# Autodesk Inventor assembly: RR-PCSS-2021-W2M1
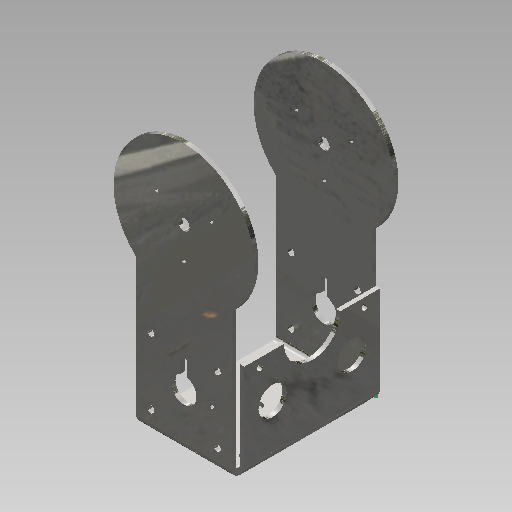
[picture p0: Inventor's stored thumbnail of the model, 512x512]
Saved by Autodesk Inventor 2021 (Build 250183000, 183)
## iProperties
Created: 2021-10-12
Part Number: RR-PCSS-2021-W2M1
Document SubType Name: Assembly
Designer: marci
Mass: 985.997 g
Surface Area: 877.416 cm^2
Volume: 123.25 cm^3
Density: 8 g/cm^3
Author: marci
## Documents named in this file (3)
- C:\Users\marci\Desktop\Projekt ramienia\2M1\RR-PCSS-2021-W2M1.iam
- C:\Users\marci\Desktop\Projekt ramienia\2M1\RR-PCSS-2021-W2M1Dn.ipt
- C:\Users\marci\Desktop\Projekt ramienia\2M1\RR-PCSS-2021-WN2M1.ipt
## Components (2 placed, 2 different names)
1. RR-PCSS-2021-W2M1Dn:1 — Zestawiające:1, Zestawiające:2, Równoległe:1
2. RR-PCSS-2021-WN2M1:1 — Zestawiające:1, Zestawiające:2, Równoległe:1
## Relationships (3: Mate 2, Flush 1)
- Zestawiające:1 [Mate]: RR-PCSS-2021-W2M1Dn:1 ↔ RR-PCSS-2021-WN2M1:1
- Zestawiające:2 [Mate] (3 mm): RR-PCSS-2021-W2M1Dn:1 ↔ RR-PCSS-2021-WN2M1:1
- Równoległe:1 [Flush] (3 mm): RR-PCSS-2021-W2M1Dn:1 ↔ RR-PCSS-2021-WN2M1:1
